# Autodesk Inventor assembly: brushless_20
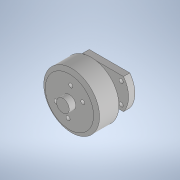
[picture p0: Inventor's stored thumbnail of the model, 180x180]
Saved by Autodesk Inventor 2020 (Build 240168000, 168)
## iProperties
Created: 2020-08-02
Part Number: brushless_20
Document SubType Name: Assembly
Designer: psrobotics
Author: psrobotics
## Documents named in this file (3)
- F:\projects-3\smartcar_3\hardware\ver1\brushless_20.iam
- F:\projects-3\smartcar_3\hardware\ver1\burshless_20_base.ipt
- F:\projects-3\smartcar_3\hardware\ver1\burshless_20_top.ipt
## Components (2 placed, 2 different names)
1. burshless_20_base:1 — Insert:1
2. burshless_20_top:1 — Insert:1
## Relationships (1: Insert 1)
- Insert:1: burshless_20_base:1 ↔ burshless_20_top:1
